# Autodesk Inventor assembly: 305-U
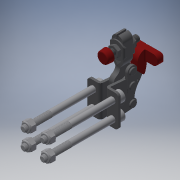
[picture p0: Inventor's stored thumbnail of the model, 180x180]
Saved by Autodesk Inventor 2018 (Build 220112000, 112)
## iProperties
Category: PARTsolutions
Company: DESTACO
Created: 2018-01-28
Part Number: 305-U
Catalog Web Link: www.cadenas.de
Description: 305-U, 307-U, 309-U-compact clamps
Vendor: DESTACO
Document SubType Name: Assembly
Designer: psAdmin
Manufacturer: DESTACO
PSOL_IDENT_0: {$CADENAS_DATA\23d-libs\destaco\destaco_gmbh\man_spann\horizontalspanner\kompakt\u_komp_assmtab.prj}
PSOL_IDENT_1: ,173 {VTYP=3D},{STYP=ASSTAB},{NB=305-U},{LINA=305-U},{NN=305-U, 307-U, 309-U},{DATE=20.09.2016 07:53
PSOL_IDENT_2: :11},{GEOMDATE=30.11.2011},{VERSION=v1},{LINEID=320},{LINESUBID=-1},{WBVAR=}  {NB=305-U},{LINA=305-U
PSOL_IDENT_3: },{KT=DUMMY},{MODELL=305-U},{HALTEKRAFT=650},{OEFFNUNG=90°},{GEWICHT=0.06kg [0.13lb]},{ANDRUCKSPINDE
PSOL_IDENT_4: L=305208-M},{A=13.5},{A1=26.0},{A3=6.4},{B=16.0},{B1=25.5},{C=12.6},{C1=8.0},{C2=2.0},{D=4.6},{F=5.4
PSOL_IDENT_5: },{H=37.0},{L=56.2},{L1=30.2},{L2=12.9},{L3=12.8},{M=M5},{SIZE=1},{MOD=1.000},{PPATH=u_kompakt_assem
PSOL_IDENT_6: blies/u_komp_sbl.prj}
NN: 305-U, 307-U, 309-U
NT: compact clamps
NB: 305-U
NBSYN: $MODELL.
LINA: 305-U
MODELL: 305-U
HALTEKRAFT: 650
OEFFNUNG: 90°
GEWICHT: 0.06kg [0.13lb]
ANDRUCKSPINDEL: 305208-M
A: 13.5
A1: 26.0
A3: 6.4
B: 16.0
B1: 25.5
C: 12.6
C1: 8.0
C2: 2.0
D: 4.6
F: 5.4
H: 37.0
L: 56.2
L1: 30.2
L2: 12.9
L3: 12.8
M: M5
SUPPLIER: DESTACO
ARTICLENO: 305-U
BOMINFO: 305-U
CREATOR: CADENAS GmbH
Title: 305-U
Author: Cadenas PARTsolutions
Comments: compact clamps
## Documents named in this file (9)
- C:\Users\maste\OneDrive\Documents\GitHub\2019CAD\Summer Drivebase\Drivebase PowerUp Files\AIS2018\305-U.iam
- C:\Users\maste\OneDrive\Documents\GitHub\2019CAD\Summer Drivebase\Drivebase PowerUp Files\AIS2018\305-U-W.ipt
- C:\Users\maste\OneDrive\Documents\GitHub\2019CAD\Summer Drivebase\Drivebase PowerUp Files\AIS2018\305104_105.ipt
- C:\Users\maste\OneDrive\Documents\GitHub\2019CAD\Summer Drivebase\Drivebase PowerUp Files\AIS2018\305106_7-KOMP.ipt
- C:\Users\maste\OneDrive\Documents\GitHub\2019CAD\Summer Drivebase\Drivebase PowerUp Files\AIS2018\305103-M-KOMP.ipt
- C:\Users\maste\OneDrive\Documents\GitHub\2019CAD\Summer Drivebase\Drivebase PowerUp Files\AIS2018\102111-M-KOMP.ipt
- C:\Users\maste\OneDrive\Documents\GitHub\2019CAD\Summer Drivebase\Drivebase PowerUp Files\AIS2018\305208-KOMP.ipt
- C:\Users\maste\OneDrive\Documents\GitHub\2019CAD\Drivebase but Calvin is a mad man\91292A197_TYPE 18-8 SS SOCKET HEAD CAP SCREW (1).ipt
- C:\Users\maste\OneDrive\Documents\GitHub\2019CAD\Drivebase but Calvin is a mad man\93625A200_TYPE 18-8 STAINLESS STL NYLON-INSERT LOCKNUT.ipt
## Components (15 placed, 8 different names)
1. 305-U-W:1 — Mate:1, Mate:2, Mate:3, Mate:4, Mate:5, Mate:6, Mate:7, Mate:8, Mate:13, Mate:14, Mate:15, Mate:16
2. 305104_105:1
3. 305106_7-KOMP:1
4. 305103-M-KOMP:1
5. 102111-M-KOMP:1
6. 102111-M-KOMP:2
7. 305208-KOMP:1
8. 91292A197_TYPE 18-8 SS SOCKET HEAD CAP SCREW (1):1 — Mate:4, Mate:5, Mate:11
9. 91292A197_TYPE 18-8 SS SOCKET HEAD CAP SCREW (1):2 — Mate:2, Mate:8, Mate:12
10. 91292A197_TYPE 18-8 SS SOCKET HEAD CAP SCREW (1):3 — Mate:1, Mate:6, Mate:9
11. 91292A197_TYPE 18-8 SS SOCKET HEAD CAP SCREW (1):4 — Mate:3, Mate:7, Mate:10
12. 93625A200_TYPE 18-8 STAINLESS STL NYLON-INSERT LOCKNUT:1 — Mate:12, Mate:13
13. 93625A200_TYPE 18-8 STAINLESS STL NYLON-INSERT LOCKNUT:2 — Mate:11, Mate:16
14. 93625A200_TYPE 18-8 STAINLESS STL NYLON-INSERT LOCKNUT:3 — Mate:10, Mate:15
15. 93625A200_TYPE 18-8 STAINLESS STL NYLON-INSERT LOCKNUT:4 — Mate:9, Mate:14
## Relationships (16: Mate 16)
- Mate:1: 305-U-W:1 ↔ 91292A197_TYPE 18-8 SS SOCKET HEAD CAP SCREW (1):3
- Mate:2: 305-U-W:1 ↔ 91292A197_TYPE 18-8 SS SOCKET HEAD CAP SCREW (1):2
- Mate:3: 305-U-W:1 ↔ 91292A197_TYPE 18-8 SS SOCKET HEAD CAP SCREW (1):4
- Mate:4: 305-U-W:1 ↔ 91292A197_TYPE 18-8 SS SOCKET HEAD CAP SCREW (1):1
- Mate:5: 305-U-W:1 ↔ 91292A197_TYPE 18-8 SS SOCKET HEAD CAP SCREW (1):1
- Mate:6: 305-U-W:1 ↔ 91292A197_TYPE 18-8 SS SOCKET HEAD CAP SCREW (1):3
- Mate:7: 305-U-W:1 ↔ 91292A197_TYPE 18-8 SS SOCKET HEAD CAP SCREW (1):4
- Mate:8: 305-U-W:1 ↔ 91292A197_TYPE 18-8 SS SOCKET HEAD CAP SCREW (1):2
- Mate:9: 91292A197_TYPE 18-8 SS SOCKET HEAD CAP SCREW (1):3 ↔ 93625A200_TYPE 18-8 STAINLESS STL NYLON-INSERT LOCKNUT:4
- Mate:10: 91292A197_TYPE 18-8 SS SOCKET HEAD CAP SCREW (1):4 ↔ 93625A200_TYPE 18-8 STAINLESS STL NYLON-INSERT LOCKNUT:3
- Mate:11: 91292A197_TYPE 18-8 SS SOCKET HEAD CAP SCREW (1):1 ↔ 93625A200_TYPE 18-8 STAINLESS STL NYLON-INSERT LOCKNUT:2
- Mate:12: 91292A197_TYPE 18-8 SS SOCKET HEAD CAP SCREW (1):2 ↔ 93625A200_TYPE 18-8 STAINLESS STL NYLON-INSERT LOCKNUT:1
- Mate:13 (50.8 mm): 305-U-W:1 ↔ 93625A200_TYPE 18-8 STAINLESS STL NYLON-INSERT LOCKNUT:1
- Mate:14 (50.8 mm): 305-U-W:1 ↔ 93625A200_TYPE 18-8 STAINLESS STL NYLON-INSERT LOCKNUT:4
- Mate:15 (50.8 mm): 305-U-W:1 ↔ 93625A200_TYPE 18-8 STAINLESS STL NYLON-INSERT LOCKNUT:3
- Mate:16 (50.8 mm): 305-U-W:1 ↔ 93625A200_TYPE 18-8 STAINLESS STL NYLON-INSERT LOCKNUT:2
